# Autodesk Inventor assembly: Cheb. korp
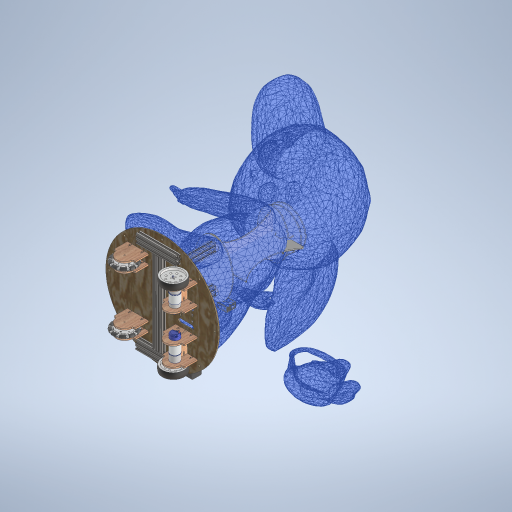
[picture p0: Inventor's stored thumbnail of the model, 512x512]
Saved by Autodesk Inventor 2023.1 (Build 271208000, 208)
## iProperties
Created: 2023-03-13
Part Number: Cheb. korp
Document SubType Name: Assembly
Designer: User
Author: User
## Documents named in this file (32)
- C:\Users\DELL\Desktop\Cheburashka_construction\Cheburashka\cheb\Cheb. korp.iam
- C:\Users\DELL\Desktop\Cheburashka_construction\Cheburashka\cheb\Osn. platform.ipt
- C:\Users\DELL\Desktop\Cheburashka_construction\Cheburashka\cheb\motor1.ipt
- C:\Users\DELL\Desktop\Cheburashka_construction\Cheburashka\cheb\motor2.ipt
- C:\Users\DELL\Desktop\Cheburashka_construction\Cheburashka\cheb\motor3.ipt
- C:\Users\DELL\Desktop\Cheburashka_construction\Cheburashka\cheb\wheel1.ipt
- C:\Users\DELL\Desktop\Cheburashka_construction\Cheburashka\cheb\Импорт\44260_txm torquenado dc motor_MIR2.ipt
- C:\Users\DELL\Desktop\Cheburashka_construction\Cheburashka\cheb\Импорт\36466_txm-4 inch omni wheel.ipt
- C:\Users\DELL\Desktop\Cheburashka_construction\Cheburashka\cheb\Импорт\39055_txm-4 inch wheel_MIR1.ipt
- C:\Users\DELL\Desktop\Cheburashka_construction\Cheburashka\cheb\motor1_MIR3.ipt
- C:\Users\DELL\Desktop\Cheburashka_construction\Cheburashka\cheb\motor2_MIR3.ipt
- C:\Users\DELL\Desktop\Cheburashka_construction\Cheburashka\cheb\motor3_MIR3.ipt
- C:\Users\DELL\Desktop\Cheburashka_construction\Cheburashka\cheb\Импорт\44260_txm torquenado dc motor_MIR2_MIR.ipt
- C:\Users\DELL\Desktop\Cheburashka_construction\Cheburashka\cheb\wheel1_MIR.ipt
- C:\Users\DELL\Desktop\Cheburashka_construction\Cheburashka\cheb\Импорт\36466_txm-4 inch omni wheel_MIR2.ipt
- C:\Users\DELL\Desktop\Cheburashka_construction\Cheburashka\cheb\Импорт\39055_txm-4 inch wheel_MIR1_MIR.ipt
- C:\Users\DELL\Desktop\Cheburashka_construction\Cheburashka\cheb\image.ipt
- C:\Users\DELL\Desktop\Cheburashka_construction\Cheburashka\cheb\Импорт\224HX-Konstruktsionnyy-profil-20kh20H.iam
- C:\Users\DELL\Desktop\Cheburashka_construction\Cheburashka\cheb\Импорт\нижний эллипс тела.ipt
- C:\Users\DELL\Desktop\Cheburashka_construction\Cheburashka\cheb\Импорт\грань тела.ipt
- C:\Users\DELL\Desktop\Cheburashka_construction\Cheburashka\cheb\Импорт\верхний эллипс туловища.ipt
- C:\Users\DELL\Desktop\Cheburashka_construction\Cheburashka\cheb\Импорт\нижний эллипс головы.ipt
- C:\Users\DELL\Desktop\Cheburashka_construction\Cheburashka\cheb\Импорт\опорная окружность.ipt
- C:\Users\DELL\Desktop\Cheburashka_construction\Cheburashka\cheb\Импорт\Servo.ipt
- C:\Users\DELL\Desktop\Cheburashka_construction\Cheburashka\cheb\Импорт\крепление шеи1.ipt
- C:\Users\DELL\Downloads\Pitsco Education-739028.ipt
- C:\Users\DELL\Desktop\Cheburashka_construction\Cheburashka\cheb\Импорт\Pitsco Education-739085.ipt
- C:\Users\DELL\Desktop\Cheburashka_construction\Cheburashka\cheb\трубка.ipt
- C:\Users\DELL\Desktop\Cheburashka_construction\Cheburashka\cheb\Импорт\Prostavka.ipt
- C:\Users\DELL\Desktop\Cheburashka_construction\Cheburashka\cheb\Деталь2.ipt
- C:\Users\DELL\Desktop\Cheburashka_construction\Cheburashka\cheb\лицо1.ipt
- C:\Users\DELL\Desktop\Cheburashka_construction\Cheburashka\cheb\Импорт\ImageToStl.com_de33b05f-b2d7-4424-b04b-15da999b358a.ipt
## Components (42 placed, 31 different names)
1. image:1
2. Osn. platform:1 — Совмещение:1, Совмещение:2, Совмещение:5, Совмещение:8, Совмещение:13, Совмещение:17, Совмещение:29, Совмещение:30, Совмещение:31, Совмещение:32, Совмещение:33, Совмещение:34, Совмещение:35, Совмещение:36, Совмещение:37, Совмещение:38, Заподлицо:2, Совмещение:45, Совмещение:46, Заподлицо:3, Совмещение:47, Совмещение:48, Совмещение:49, Совмещение:50, Совмещение:51, Совмещение:53, Заподлицо:4
3. motor1:1 — Совмещение:2, Совмещение:31, Совмещение:32
4. motor2:1 — Совмещение:5, Совмещение:29, Совмещение:30
5. motor3:1 — Совмещение:8, Совмещение:11, Совмещение:12, Совмещение:22, Совмещение:33, Совмещение:34
6. 44260_txm torquenado dc motor_MIR2:1 — Совмещение:11, Совмещение:12, Совмещение:21
7. wheel1:1 — Совмещение:13, Совмещение:19, Совмещение:20, Совмещение:37, Совмещение:38
8. wheel1:2 — Совмещение:17, Совмещение:35, Совмещение:36
9. 36466_txm-4 inch omni wheel:1 — Совмещение:19, Совмещение:20
10. 39055_txm-4 inch wheel_MIR1:1 — Совмещение:21, Совмещение:22
11. motor1_MIR3:1
12. motor2_MIR3:1
13. motor3_MIR3:1 — Совмещение:23, Совмещение:24, Совмещение:27
14. 44260_txm torquenado dc motor_MIR2_MIR:1 — Совмещение:23, Совмещение:24, Совмещение:28
15. wheel1_MIR:1 — Совмещение:25, Совмещение:26
16. wheel1_MIR:2
17. 36466_txm-4 inch omni wheel_MIR2:1 — Совмещение:25, Совмещение:26
18. 39055_txm-4 inch wheel_MIR1_MIR:1 — Совмещение:27, Совмещение:28
19. 224HX-Konstruktsionnyy-profil-20kh20H:1 [sub-assembly] — Заподлицо:2, Совмещение:45, Совмещение:46
20. 224HX-Konstruktsionnyy-profil-20kh20H:3 [sub-assembly] — Совмещение:49, Совмещение:50, Совмещение:52, Совмещение:54
21. 224HX-Konstruktsionnyy-profil-20kh20H:4 [sub-assembly] — Заподлицо:3, Совмещение:47, Совмещение:48
22. 224HX-Konstruktsionnyy-profil-20kh20H:5 [sub-assembly] — Совмещение:51, Совмещение:52
23. 224HX-Konstruktsionnyy-profil-20kh20H:6 [sub-assembly] — Совмещение:53, Совмещение:54
24. нижний эллипс тела:1 — Заподлицо:5, Заподлицо:6, Совмещение:82
25. грань тела:1 — Заподлицо:6, Заподлицо:8, Совмещение:61, Угол:1
26. верхний эллипс туловища:1 — Заподлицо:8, Заподлицо:9, Совмещение:66, Совмещение:67, Совмещение:69
27. нижний эллипс головы:1 — Заподлицо:10, Заподлицо:11, Совмещение:73
28. опорная окружность:1 — Заподлицо:12
29. Servo:1
30. Servo:2
31. Servo:3
32. крепление шеи1:1 — Совмещение:61
33. Pitsco Education-739028:1 — Совмещение:78, Совмещение:79
34. Pitsco Education-739085:1 — Совмещение:68, Совмещение:75, Совмещение:80
35. трубка:1 — Совмещение:66, Совмещение:67, Совмещение:68, Совмещение:74, Совмещение:81
36. Servo:4 — Совмещение:69, Совмещение:76, Совмещение:77
37. Prostavka:1 — Совмещение:73, Совмещение:74, Совмещение:75
38. Деталь2:1 — Совмещение:76, Совмещение:77, Совмещение:78, Совмещение:79
39. Prostavka:2 — Совмещение:80, Совмещение:81, Заподлицо:16
40. лицо1:1 — Заподлицо:16
41. грань тела:2 — Угол:1, Совмещение:82
42. ImageToStl.com_de33b05f-b2d7-4424-b04b-15da999b358a:1
## Relationships (65: Mate 53, Flush 11, Angle 1)
- Совмещение:1 [Mate]: Osn. platform:1
- Совмещение:2 [Mate]: Osn. platform:1 ↔ motor1:1
- Совмещение:5 [Mate]: Osn. platform:1 ↔ motor2:1
- Совмещение:8 [Mate]: Osn. platform:1 ↔ motor3:1
- Совмещение:11 [Mate]: motor3:1 ↔ 44260_txm torquenado dc motor_MIR2:1
- Совмещение:12 [Mate]: motor3:1 ↔ 44260_txm torquenado dc motor_MIR2:1
- Совмещение:13 [Mate]: Osn. platform:1 ↔ wheel1:1
- Совмещение:17 [Mate]: Osn. platform:1 ↔ wheel1:2
- Совмещение:19 [Mate]: wheel1:1 ↔ 36466_txm-4 inch omni wheel:1
- Совмещение:20 [Mate] (10 mm): wheel1:1 ↔ 36466_txm-4 inch omni wheel:1
- Совмещение:21 [Mate]: 44260_txm torquenado dc motor_MIR2:1 ↔ 39055_txm-4 inch wheel_MIR1:1
- Совмещение:22 [Mate] (15 mm): motor3:1 ↔ 39055_txm-4 inch wheel_MIR1:1
- Совмещение:23 [Mate]: motor3_MIR3:1 ↔ 44260_txm torquenado dc motor_MIR2_MIR:1
- Совмещение:24 [Mate]: motor3_MIR3:1 ↔ 44260_txm torquenado dc motor_MIR2_MIR:1
- Совмещение:25 [Mate] (10 mm): wheel1_MIR:1 ↔ 36466_txm-4 inch omni wheel_MIR2:1
- Совмещение:26 [Mate]: wheel1_MIR:1 ↔ 36466_txm-4 inch omni wheel_MIR2:1
- Совмещение:27 [Mate] (15 mm): motor3_MIR3:1 ↔ 39055_txm-4 inch wheel_MIR1_MIR:1
- Совмещение:28 [Mate]: 44260_txm torquenado dc motor_MIR2_MIR:1 ↔ 39055_txm-4 inch wheel_MIR1_MIR:1
- Совмещение:29 [Mate]: Osn. platform:1 ↔ motor2:1
- Совмещение:30 [Mate]: Osn. platform:1 ↔ motor2:1
- Совмещение:31 [Mate]: Osn. platform:1 ↔ motor1:1
- Совмещение:32 [Mate]: Osn. platform:1 ↔ motor1:1
- Совмещение:33 [Mate]: Osn. platform:1 ↔ motor3:1
- Совмещение:34 [Mate]: Osn. platform:1 ↔ motor3:1
- Совмещение:35 [Mate]: Osn. platform:1 ↔ wheel1:2
- Совмещение:36 [Mate]: Osn. platform:1 ↔ wheel1:2
- Совмещение:37 [Mate]: Osn. platform:1 ↔ wheel1:1
- Совмещение:38 [Mate]: Osn. platform:1 ↔ wheel1:1
- Заподлицо:2 [Flush]: Osn. platform:1 ↔ 224HX-Konstruktsionnyy-profil-20kh20H:1
- Совмещение:45 [Mate]: Osn. platform:1 ↔ 224HX-Konstruktsionnyy-profil-20kh20H:1
- Совмещение:46 [Mate]: Osn. platform:1 ↔ 224HX-Konstruktsionnyy-profil-20kh20H:1
- Заподлицо:3 [Flush]: Osn. platform:1 ↔ 224HX-Konstruktsionnyy-profil-20kh20H:4
- Совмещение:47 [Mate]: Osn. platform:1 ↔ 224HX-Konstruktsionnyy-profil-20kh20H:4
- Совмещение:48 [Mate]: Osn. platform:1 ↔ 224HX-Konstruktsionnyy-profil-20kh20H:4
- Совмещение:49 [Mate]: Osn. platform:1 ↔ 224HX-Konstruktsionnyy-profil-20kh20H:3
- Совмещение:50 [Mate]: Osn. platform:1 ↔ 224HX-Konstruktsionnyy-profil-20kh20H:3
- Совмещение:51 [Mate]: Osn. platform:1 ↔ 224HX-Konstruktsionnyy-profil-20kh20H:5
- Совмещение:52 [Mate]: 224HX-Konstruktsionnyy-profil-20kh20H:3 ↔ 224HX-Konstruktsionnyy-profil-20kh20H:5
- Совмещение:53 [Mate]: Osn. platform:1 ↔ 224HX-Konstruktsionnyy-profil-20kh20H:6
- Совмещение:54 [Mate]: 224HX-Konstruktsionnyy-profil-20kh20H:3 ↔ 224HX-Konstruktsionnyy-profil-20kh20H:6
- Заподлицо:4 [Flush] (230 mm): Osn. platform:1
- Заподлицо:5 [Flush]: нижний эллипс тела:1
- Заподлицо:6 [Flush]: нижний эллипс тела:1 ↔ грань тела:1
- Заподлицо:8 [Flush]: грань тела:1 ↔ верхний эллипс туловища:1
- Заподлицо:9 [Flush] (40 mm): верхний эллипс туловища:1
- Заподлицо:10 [Flush]: нижний эллипс головы:1
- Заподлицо:11 [Flush] (20 mm): нижний эллипс головы:1
- Заподлицо:12 [Flush]: опорная окружность:1
- Совмещение:61 [Mate]: грань тела:1 ↔ крепление шеи1:1
- Совмещение:66 [Mate]: верхний эллипс туловища:1 ↔ трубка:1
- Совмещение:67 [Mate]: верхний эллипс туловища:1 ↔ трубка:1
- Совмещение:68 [Mate]: Pitsco Education-739085:1 ↔ трубка:1
- Совмещение:69 [Mate]: верхний эллипс туловища:1 ↔ Servo:4
- Совмещение:73 [Mate]: нижний эллипс головы:1 ↔ Prostavka:1
- Совмещение:74 [Mate]: трубка:1 ↔ Prostavka:1
- Совмещение:75 [Mate]: Pitsco Education-739085:1 ↔ Prostavka:1
- Совмещение:76 [Mate]: Servo:4 ↔ Деталь2:1
- Совмещение:77 [Mate]: Servo:4 ↔ Деталь2:1
- Совмещение:78 [Mate]: Pitsco Education-739028:1 ↔ Деталь2:1
- Совмещение:79 [Mate]: Pitsco Education-739028:1 ↔ Деталь2:1
- Совмещение:80 [Mate]: Pitsco Education-739085:1 ↔ Prostavka:2
- Совмещение:81 [Mate]: трубка:1 ↔ Prostavka:2
- Заподлицо:16 [Flush]: Prostavka:2 ↔ лицо1:1
- Угол:1 [Angle] (90 deg): грань тела:1 ↔ грань тела:2
- Совмещение:82 [Mate]: нижний эллипс тела:1 ↔ грань тела:2
